# Autodesk Inventor assembly: Assembly1
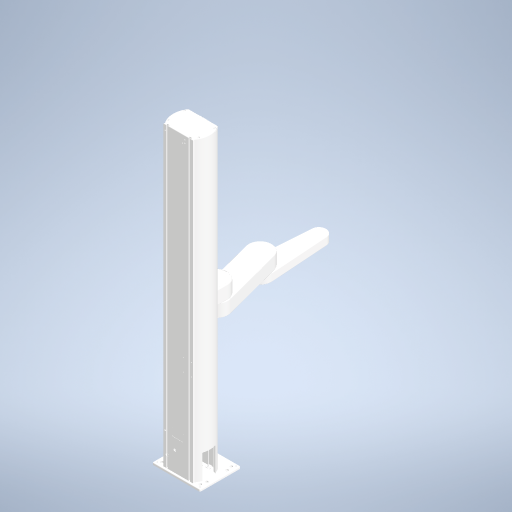
[picture p0: Inventor's stored thumbnail of the model, 512x512]
Saved by Autodesk Inventor 2023 (Build 270158000, 158)
## iProperties
Created: 2022-09-20
Part Number: Assembly1
Document SubType Name: Assembly
Designer: benni
Author: benni
## Documents named in this file (5)
- C:\Users\benni\Documents\Studium\7. Semester\Industrial Robotics\Assignment 2\@PF3400\CAD\OldVersions\Assembly1.iam
- C:\Users\benni\Documents\Studium\7. Semester\Industrial Robotics\Assignment 2\@PF3400\CAD\Base.ipt
- C:\Users\benni\Documents\Studium\7. Semester\Industrial Robotics\Assignment 2\@PF3400\CAD\Carriage.ipt
- C:\Users\benni\Documents\Studium\7. Semester\Industrial Robotics\Assignment 2\@PF3400\CAD\InnerArm.ipt
- C:\Users\benni\Documents\Studium\7. Semester\Industrial Robotics\Assignment 2\@PF3400\CAD\OuterArm.ipt
## Components (4 placed, 4 different names)
1. Base:1 — Mate:1, Flush:1, Mate:2, Flush:2, Flush:3
2. Carriage:1 — Flush:2, Flush:3, Insert:1
3. InnerArm:1 — Insert:1, Insert:2
4. OuterArm:1 — Insert:2
## Relationships (7: Flush 3, Mate 2, Insert 2)
- Mate:1: Base:1
- Flush:1: Base:1
- Mate:2: Base:1
- Flush:2: Base:1 ↔ Carriage:1
- Flush:3: Base:1 ↔ Carriage:1
- Insert:1: Carriage:1 ↔ InnerArm:1
- Insert:2: InnerArm:1 ↔ OuterArm:1
